# Autodesk Inventor assembly: Cuadrúpedo - Ensamble 3 DOF
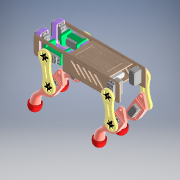
[picture p0: Inventor's stored thumbnail of the model, 180x180]
Saved by Autodesk Inventor 2019 (Build 230136000, 136)
## iProperties
Created: 2020-03-12
Part Number: Cuadrúpedo - Ensamble 3 DOF
Document SubType Name: Assembly
Designer: Sanoli
Author: Sanoli
## Documents named in this file (13)
- E:\Escritorio\Temporal\Documentos\Robótica I\Proyectos\Cuadrúpedo\Diseño Mecánico\Cuadrúpedo - Ensamble 3 DOF.iam
- E:\Escritorio\Temporal\Documentos\Robótica I\Proyectos\Cuadrúpedo\Diseño Mecánico\Cuerpo - Base Batería.ipt
- E:\Escritorio\Temporal\Documentos\Robótica I\Proyectos\Cuadrúpedo\Diseño Mecánico\Cuerpo - Acople Hombro.ipt
- E:\Escritorio\Temporal\Documentos\Robótica I\Proyectos\Cuadrúpedo\Diseño Mecánico\Cuerpo - Batería.ipt
- E:\Escritorio\Temporal\Documentos\Robótica I\Proyectos\Cuadrúpedo\Diseño Mecánico\Servo MG996R\Servo MG996R - Ensamble - Sin Flor.iam
- E:\Escritorio\Temporal\Documentos\Robótica I\Proyectos\Cuadrúpedo\Diseño Mecánico\Pata - Antebrazo.ipt
- E:\Escritorio\Temporal\Documentos\Robótica I\Proyectos\Cuadrúpedo\Diseño Mecánico\Servo MG996R\TowerPro SG5010 - Acople Hélice.ipt
- E:\Escritorio\Temporal\Documentos\Robótica I\Proyectos\Cuadrúpedo\Diseño Mecánico\Pata - Brazo - Pata Ninjaflex.ipt
- E:\Escritorio\Temporal\Documentos\Robótica I\Proyectos\Cuadrúpedo\Diseño Mecánico\Pata - Pie - Textura.ipt
- E:\Escritorio\Temporal\Documentos\Robótica I\Proyectos\Cuadrúpedo\Diseño Mecánico\Pata - Hombro.ipt
- E:\Escritorio\Temporal\Documentos\Robótica I\Proyectos\Cuadrúpedo\Diseño Mecánico\Cuerpo - Lateral.ipt
- E:\Escritorio\Temporal\Documentos\Robótica I\Proyectos\Cuadrúpedo\Diseño Mecánico\Cuerpo - Base Arduino.ipt
- E:\Escritorio\Temporal\Documentos\Robótica I\Proyectos\Cuadrúpedo\Diseño Mecánico\Pata - Hombro Mirror.ipt
## Components (40 placed, 12 different names)
1. Cuerpo - Base Batería:1 — Mate:1, Flush:1, Flush:2, Mate:2, Flush:3, Tangent:1, Flush:7, Mate:25, Mate:26, Flush:10, Mate:43, Mate:44
2. Cuerpo - Acople Hombro:1 — Mate:1, Flush:1, Flush:2, Mate:18, Mate:19, Mate:20, Mate:21, Mate:76, Mate:77, Mate:78, Mate:84
3. Cuerpo - Batería:1 — Mate:2, Flush:3, Tangent:1
4. Servo MG996R - Ensamble - Sin Flor:1 [sub-assembly] — Mate:22, Mate:23, Mate:24
5. Pata - Antebrazo:1
6. TowerPro SG5010 - Acople Hélice:1
7. TowerPro SG5010 - Acople Hélice:2
8. Servo MG996R - Ensamble - Sin Flor:2 [sub-assembly]
9. Pata - Brazo - Pata Ninjaflex:1
10. Pata - Pie - Textura:1
11. Servo MG996R - Ensamble - Sin Flor:3 [sub-assembly] — Mate:18, Mate:19, Mate:20
12. TowerPro SG5010 - Acople Hélice:3
13. Pata - Hombro:1 — Mate:21, Mate:22, Mate:23, Mate:24
14. Cuerpo - Lateral:2 — Flush:7, Mate:25, Mate:26, Mate:27, Mate:28, Mate:29, Mate:45
15. Servo MG996R - Ensamble - Sin Flor:4 [sub-assembly] — Mate:27, Mate:28, Mate:29, Flush:9, Mate:42
16. Pata - Antebrazo:2
17. TowerPro SG5010 - Acople Hélice:4
18. TowerPro SG5010 - Acople Hélice:5 — Flush:9, Mate:42
19. Servo MG996R - Ensamble - Sin Flor:5 [sub-assembly]
20. Pata - Brazo - Pata Ninjaflex:2
21. Pata - Pie - Textura:2
22. Cuerpo - Lateral:3 — Flush:10, Mate:43, Mate:44, Flush:11, Mate:46, Mate:60, Mate:61, Mate:62
23. Cuerpo - Base Arduino:1 — Mate:45, Flush:11, Mate:46
24. Servo MG996R - Ensamble - Sin Flor:6 [sub-assembly] — Mate:60, Mate:61, Mate:62
25. TowerPro SG5010 - Acople Hélice:6
26. Pata - Antebrazo:3
27. TowerPro SG5010 - Acople Hélice:7
28. Pata - Brazo - Pata Ninjaflex:3
29. Servo MG996R - Ensamble - Sin Flor:7 [sub-assembly]
30. Pata - Pie - Textura:3
31. Servo MG996R - Ensamble - Sin Flor:8 [sub-assembly] — Mate:85, Mate:86, Mate:87, Mate:88
32. TowerPro SG5010 - Acople Hélice:8
33. Pata - Antebrazo:4
34. TowerPro SG5010 - Acople Hélice:9
35. Pata - Brazo - Pata Ninjaflex:4
36. Servo MG996R - Ensamble - Sin Flor:9 [sub-assembly]
37. Pata - Pie - Textura:4
38. Pata - Hombro Mirror:1 — Mate:79, Mate:80, Mate:81, Mate:82, Mate:84, Mate:85, Mate:86, Mate:87, Mate:88
39. Servo MG996R - Ensamble - Sin Flor:10 [sub-assembly] — Mate:76, Mate:77, Mate:78, Mate:83
40. TowerPro SG5010 - Acople Hélice:11 — Mate:79, Mate:80, Mate:81, Mate:82, Mate:83
## Relationships (104: Mate 88, Flush 15, Tangent 1)
- Mate:1: Cuerpo - Base Batería:1 ↔ Cuerpo - Acople Hombro:1
- Flush:1: Cuerpo - Base Batería:1 ↔ Cuerpo - Acople Hombro:1
- Flush:2: Cuerpo - Base Batería:1 ↔ Cuerpo - Acople Hombro:1
- Mate:2: Cuerpo - Base Batería:1 ↔ Cuerpo - Batería:1
- Flush:3: Cuerpo - Base Batería:1 ↔ Cuerpo - Batería:1
- Tangent:1: Cuerpo - Base Batería:1 ↔ Cuerpo - Batería:1
- [Mate]: Pata - Antebrazo:1 ↔ TowerPro SG5010 - Acople Hélice:2
- [Mate]: Pata - Antebrazo:1 ↔ TowerPro SG5010 - Acople Hélice:2
- [Mate]: Pata - Antebrazo:1 ↔ TowerPro SG5010 - Acople Hélice:2
- [Mate]: Pata - Antebrazo:1 ↔ TowerPro SG5010 - Acople Hélice:1
- [Mate]: Pata - Antebrazo:1 ↔ TowerPro SG5010 - Acople Hélice:1
- [Mate]: Pata - Antebrazo:1 ↔ TowerPro SG5010 - Acople Hélice:1
- [Flush]: Servo MG996R - Ensamble - Sin Flor:1 ↔ TowerPro SG5010 - Acople Hélice:2
- [Mate]: Servo MG996R - Ensamble - Sin Flor:1 ↔ TowerPro SG5010 - Acople Hélice:2
- [Mate]: Pata - Brazo - Pata Ninjaflex:1 ↔ Pata - Pie - Textura:1
- [Mate]: Pata - Brazo - Pata Ninjaflex:1 ↔ Pata - Pie - Textura:1
- [Mate]: Servo MG996R - Ensamble - Sin Flor:2 ↔ Pata - Brazo - Pata Ninjaflex:1
- [Mate]: Servo MG996R - Ensamble - Sin Flor:2 ↔ Pata - Brazo - Pata Ninjaflex:1
- [Mate]: Servo MG996R - Ensamble - Sin Flor:2 ↔ Pata - Brazo - Pata Ninjaflex:1
- [Flush]: TowerPro SG5010 - Acople Hélice:1 ↔ Servo MG996R - Ensamble - Sin Flor:2
- [Mate]: TowerPro SG5010 - Acople Hélice:1 ↔ Servo MG996R - Ensamble - Sin Flor:2
- [Flush]: Servo MG996R - Ensamble - Sin Flor:3 ↔ TowerPro SG5010 - Acople Hélice:3
- [Mate]: Servo MG996R - Ensamble - Sin Flor:3 ↔ TowerPro SG5010 - Acople Hélice:3
- [Mate]: TowerPro SG5010 - Acople Hélice:3 ↔ Pata - Hombro:1
- Mate:18: Cuerpo - Acople Hombro:1 ↔ Servo MG996R - Ensamble - Sin Flor:3
- Mate:19: Cuerpo - Acople Hombro:1 ↔ Servo MG996R - Ensamble - Sin Flor:3
- Mate:20: Cuerpo - Acople Hombro:1 ↔ Servo MG996R - Ensamble - Sin Flor:3
- Mate:21: Cuerpo - Acople Hombro:1 ↔ Pata - Hombro:1
- Mate:22: Servo MG996R - Ensamble - Sin Flor:1 ↔ Pata - Hombro:1
- Mate:23: Servo MG996R - Ensamble - Sin Flor:1 ↔ Pata - Hombro:1
- Mate:24: Servo MG996R - Ensamble - Sin Flor:1 ↔ Pata - Hombro:1
- Flush:7: Cuerpo - Base Batería:1 ↔ Cuerpo - Lateral:2
- Mate:25: Cuerpo - Base Batería:1 ↔ Cuerpo - Lateral:2
- Mate:26: Cuerpo - Base Batería:1 ↔ Cuerpo - Lateral:2
- Mate:27: Cuerpo - Lateral:2 ↔ Servo MG996R - Ensamble - Sin Flor:4
- Mate:28: Cuerpo - Lateral:2 ↔ Servo MG996R - Ensamble - Sin Flor:4
- Mate:29: Cuerpo - Lateral:2 ↔ Servo MG996R - Ensamble - Sin Flor:4
- [Mate]: Pata - Antebrazo:2 ↔ TowerPro SG5010 - Acople Hélice:5
- [Mate]: Pata - Antebrazo:2 ↔ TowerPro SG5010 - Acople Hélice:5
- [Mate]: Pata - Antebrazo:2 ↔ TowerPro SG5010 - Acople Hélice:5
- [Mate]: Pata - Antebrazo:2 ↔ TowerPro SG5010 - Acople Hélice:4
- [Mate]: Pata - Antebrazo:2 ↔ TowerPro SG5010 - Acople Hélice:4
- [Mate]: Pata - Antebrazo:2 ↔ TowerPro SG5010 - Acople Hélice:4
- [Mate]: Pata - Brazo - Pata Ninjaflex:2 ↔ Pata - Pie - Textura:2
- [Mate]: Pata - Brazo - Pata Ninjaflex:2 ↔ Pata - Pie - Textura:2
- [Mate]: Servo MG996R - Ensamble - Sin Flor:5 ↔ Pata - Brazo - Pata Ninjaflex:2
- [Mate]: Servo MG996R - Ensamble - Sin Flor:5 ↔ Pata - Brazo - Pata Ninjaflex:2
- [Mate]: Servo MG996R - Ensamble - Sin Flor:5 ↔ Pata - Brazo - Pata Ninjaflex:2
- [Flush]: TowerPro SG5010 - Acople Hélice:4 ↔ Servo MG996R - Ensamble - Sin Flor:5
- [Mate]: TowerPro SG5010 - Acople Hélice:4 ↔ Servo MG996R - Ensamble - Sin Flor:5
- Flush:9: Servo MG996R - Ensamble - Sin Flor:4 ↔ TowerPro SG5010 - Acople Hélice:5
- Mate:42: Servo MG996R - Ensamble - Sin Flor:4 ↔ TowerPro SG5010 - Acople Hélice:5
- Flush:10: Cuerpo - Base Batería:1 ↔ Cuerpo - Lateral:3
- Mate:43: Cuerpo - Base Batería:1 ↔ Cuerpo - Lateral:3
- Mate:44: Cuerpo - Base Batería:1 ↔ Cuerpo - Lateral:3
- Mate:45: Cuerpo - Lateral:2 ↔ Cuerpo - Base Arduino:1
- Flush:11: Cuerpo - Lateral:3 ↔ Cuerpo - Base Arduino:1
- Mate:46: Cuerpo - Lateral:3 ↔ Cuerpo - Base Arduino:1
- [Flush]: Servo MG996R - Ensamble - Sin Flor:6 ↔ TowerPro SG5010 - Acople Hélice:6
- [Mate]: Servo MG996R - Ensamble - Sin Flor:6 ↔ TowerPro SG5010 - Acople Hélice:6
- [Mate]: Pata - Antebrazo:3 ↔ TowerPro SG5010 - Acople Hélice:7
- [Mate]: Pata - Antebrazo:3 ↔ TowerPro SG5010 - Acople Hélice:7
- [Mate]: Pata - Antebrazo:3 ↔ TowerPro SG5010 - Acople Hélice:7
- [Mate]: Pata - Brazo - Pata Ninjaflex:3 ↔ Servo MG996R - Ensamble - Sin Flor:7
- [Mate]: Pata - Brazo - Pata Ninjaflex:3 ↔ Servo MG996R - Ensamble - Sin Flor:7
- [Mate]: Pata - Brazo - Pata Ninjaflex:3 ↔ Servo MG996R - Ensamble - Sin Flor:7
- [Flush]: TowerPro SG5010 - Acople Hélice:7 ↔ Servo MG996R - Ensamble - Sin Flor:7
- [Mate]: TowerPro SG5010 - Acople Hélice:7 ↔ Servo MG996R - Ensamble - Sin Flor:7
- [Mate]: Pata - Brazo - Pata Ninjaflex:3 ↔ Pata - Pie - Textura:3
- [Mate]: Pata - Brazo - Pata Ninjaflex:3 ↔ Pata - Pie - Textura:3
- [Mate]: TowerPro SG5010 - Acople Hélice:6 ↔ Pata - Antebrazo:3
- [Mate]: Servo MG996R - Ensamble - Sin Flor:6 ↔ Pata - Antebrazo:3
- [Mate]: TowerPro SG5010 - Acople Hélice:6 ↔ Pata - Antebrazo:3
- Mate:60: Cuerpo - Lateral:3 ↔ Servo MG996R - Ensamble - Sin Flor:6
- Mate:61: Cuerpo - Lateral:3 ↔ Servo MG996R - Ensamble - Sin Flor:6
- Mate:62: Cuerpo - Lateral:3 ↔ Servo MG996R - Ensamble - Sin Flor:6
- [Flush]: Servo MG996R - Ensamble - Sin Flor:8 ↔ TowerPro SG5010 - Acople Hélice:8
- [Mate]: Servo MG996R - Ensamble - Sin Flor:8 ↔ TowerPro SG5010 - Acople Hélice:8
- [Mate]: Pata - Antebrazo:4 ↔ TowerPro SG5010 - Acople Hélice:9
- [Mate]: Pata - Antebrazo:4 ↔ TowerPro SG5010 - Acople Hélice:9
- [Mate]: Pata - Antebrazo:4 ↔ TowerPro SG5010 - Acople Hélice:9
- [Mate]: Pata - Brazo - Pata Ninjaflex:4 ↔ Servo MG996R - Ensamble - Sin Flor:9
- [Mate]: Pata - Brazo - Pata Ninjaflex:4 ↔ Servo MG996R - Ensamble - Sin Flor:9
- [Mate]: Pata - Brazo - Pata Ninjaflex:4 ↔ Servo MG996R - Ensamble - Sin Flor:9
- [Flush]: TowerPro SG5010 - Acople Hélice:9 ↔ Servo MG996R - Ensamble - Sin Flor:9
- [Mate]: TowerPro SG5010 - Acople Hélice:9 ↔ Servo MG996R - Ensamble - Sin Flor:9
- [Mate]: Pata - Brazo - Pata Ninjaflex:4 ↔ Pata - Pie - Textura:4
- [Mate]: Pata - Brazo - Pata Ninjaflex:4 ↔ Pata - Pie - Textura:4
- [Mate]: TowerPro SG5010 - Acople Hélice:8 ↔ Pata - Antebrazo:4
- [Mate]: Servo MG996R - Ensamble - Sin Flor:8 ↔ Pata - Antebrazo:4
- [Mate]: TowerPro SG5010 - Acople Hélice:8 ↔ Pata - Antebrazo:4
- Mate:76: Cuerpo - Acople Hombro:1 ↔ Servo MG996R - Ensamble - Sin Flor:10
- Mate:77: Cuerpo - Acople Hombro:1 ↔ Servo MG996R - Ensamble - Sin Flor:10
- Mate:78: Cuerpo - Acople Hombro:1 ↔ Servo MG996R - Ensamble - Sin Flor:10
- Mate:79: Pata - Hombro Mirror:1 ↔ TowerPro SG5010 - Acople Hélice:11
- Mate:80: Pata - Hombro Mirror:1 ↔ TowerPro SG5010 - Acople Hélice:11
- Mate:81: Pata - Hombro Mirror:1 ↔ TowerPro SG5010 - Acople Hélice:11
- Mate:82: Pata - Hombro Mirror:1 ↔ TowerPro SG5010 - Acople Hélice:11
- Mate:83: Servo MG996R - Ensamble - Sin Flor:10 ↔ TowerPro SG5010 - Acople Hélice:11
- Mate:84: Cuerpo - Acople Hombro:1 ↔ Pata - Hombro Mirror:1
- Mate:85: Servo MG996R - Ensamble - Sin Flor:8 ↔ Pata - Hombro Mirror:1
- Mate:86: Servo MG996R - Ensamble - Sin Flor:8 ↔ Pata - Hombro Mirror:1
- Mate:87: Servo MG996R - Ensamble - Sin Flor:8 ↔ Pata - Hombro Mirror:1
- Mate:88: Servo MG996R - Ensamble - Sin Flor:8 ↔ Pata - Hombro Mirror:1
## Named parameters: d98_d62 = 0 mm, d99_d63 = 0 mm, d42_d87 = 0 mm, d43_d88 = 0 mm, d44_d89 = 0 mm, d45_d90 = 0 mm, d46_d91 = 0 mm, d47_d92 = 0 mm, d48_d98_d62 = 0 mm, d49_d99_d63 = 0 mm, d50_d100 = 0 mm, d51_d101 = 0 mm, d52_d102 = 0 mm, d53_d103 = 0 mm, d54_d104 = 0 mm, d64_d54 = 0 mm, d65_d55 = 0 mm, d66_d56 = 0 mm, d67_d57 = 0 mm, d68_d58 = 0 mm, d69_d59 = 0 mm, d70_d60 = 0 mm, d71_d61 = 0 mm, d72_d62 = 0 mm, d73_d63 = 0 mm, d84_d64_d54 = 0 mm, d85_d65_d55 = 0 mm, d86_d66_d56 = 0 mm, d95_d67_d57 = 0 mm, d96_d68_d58 = 0 mm, d97_d69_d59 = 0 mm, d98_d70_d60 = 0 mm, d99_d71_d61 = 0 mm, d105_d72_d62 = 0 mm, d106_d73_d63 = 0 mm, d107_d74 = 0 mm, d108_d75 = 0 mm, d109_d76 = 0 mm, d110_d49 = 0 mm, d111_d50 = 0 mm
